# Autodesk Inventor assembly: CanSat
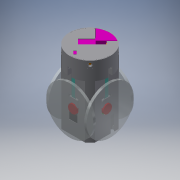
[picture p0: Inventor's stored thumbnail of the model, 180x180]
Saved by Autodesk Inventor 2018 (Build 220112000, 112)
## iProperties
Created: 2017-12-31
Part Number: CanSat
Document SubType Name: Assembly
Designer: suchanek
Author: suchanek
## Documents named in this file (19)
- C:\Users\Suchanek\Programming\CanSat\Schematics\Model\CanSat.iam
- C:\Users\Suchanek\Programming\CanSat\Schematics\Model\Hull.ipt
- C:\Users\Suchanek\Programming\CanSat\Schematics\Model\Arm.ipt
- C:\Users\Suchanek\Programming\CanSat\Schematics\Model\Motor.ipt
- C:\Users\Suchanek\Programming\CanSat\Schematics\Model\Rotor.ipt
- C:\Users\Suchanek\Programming\CanSat\Schematics\Model\Servo.ipt
- C:\Users\Suchanek\Programming\CanSat\Schematics\Model\Spring.ipt
- C:\Users\Suchanek\Programming\CanSat\Schematics\Model\Servo_bit.ipt
- C:\Users\Suchanek\Programming\CanSat\Schematics\Model\Scraper.ipt
- C:\Users\Suchanek\Programming\CanSat\Schematics\Model\Circuit.ipt
- C:\Users\Suchanek\Programming\CanSat\Schematics\Model\Flight_controler.ipt
- C:\Users\Suchanek\Programming\CanSat\Schematics\Model\HGLRC Micro 13A 4in1 BLHeli_S.ipt
- C:\Users\Suchanek\Programming\CanSat\Schematics\Model\SIM808 Module GSM GPRS GPS Breakout Board SIM808 for Arduino Raspberry.ipt
- C:\Users\Suchanek\Programming\CanSat\Schematics\Model\Motor_holder.ipt
- C:\Users\Suchanek\Programming\CanSat\Schematics\Model\Battery.ipt
- C:\Users\Suchanek\Programming\CanSat\Schematics\Model\Hull_bottom.ipt
- C:\Users\Suchanek\Programming\CanSat\Schematics\Model\Camera.ipt
- C:\Users\Suchanek\Programming\CanSat\Schematics\Model\Hull_middle.ipt
- C:\Users\Suchanek\Programming\CanSat\Schematics\Model\Hull_top.ipt
## Components (45 placed, 18 different names)
1. Hull:1 — Slider:2, Rotational:31, Flush:1, Mate:5, Mate:6, Angle:4, Mate:8, Flush:3, Mate:9, Mate:10, Cylindrical:1, Angle:5, Mate:11, Mate:12, Flush:12, Cylindrical:2, Mate:14, Mate:15, Mate:16, Mate:17, Mate:18, Flush:13, Mate:19, Mate:20, Flush:14, Mate:21, Angle:6, Flush:15, Flush:16, Mate:23, Mate:25, Mate:26
2. Servo:1 — Rotational:24, Mate:8, Flush:3, Mate:9
3. Spring:1 — Rigid:6, Rigid:7
4. Servo_bit:1 — Rotational:24, Rigid:6
5. Scraper:1 — Rigid:7
6. Circuit:1 — Mate:21, Angle:6, Flush:15, Mate:24
7. Flight_controler:1 — Cylindrical:1, Angle:5, Mate:11
8. HGLRC Micro 13A 4in1 BLHeli_S:2 — Cylindrical:2, Mate:14, Mate:15
9. SIM808 Module GSM GPRS GPS Breakout Board SIM808 for Arduino Raspberry:1 — Mate:12, Flush:12, Mate:26
10. Hull_bottom:1 — Mate:16, Mate:17, Mate:18
11. Camera:1 — Angle:4, Mate:10, Flush:13
12. Hull_middle:1 — Mate:19, Mate:20, Flush:14
13. Hull_top:1 — Flush:16, Mate:23, Mate:24, Mate:25
14. Battery:2 — Rigid:19, Rigid:20
15. Battery:1 — Rigid:18, Slider:2
16. Battery:3 — Rigid:20, Mate:5
17. Battery:4 — Rigid:18, Rigid:19, Flush:1, Mate:6
18. Battery:5
19. Battery:6
20. Battery:7
21. Battery:8
22. Battery:9
23. Battery:10
24. Battery:11
25. Battery:12
26. Battery:13
27. Battery:14
28. Battery:15
29. Battery:16
30. Arm:1 — Rotational:31, Rigid:21
31. Rotor:2 — Rotational:10
32. Motor:4 — Rotational:10, Rigid:14
33. Motor_holder:2 — Rigid:14, Rigid:21
34. Arm:2
35. Rotor:3
36. Motor:5
37. Motor_holder:3
38. Arm:3
39. Rotor:4
40. Motor:6
41. Motor_holder:4
42. Arm:4
43. Rotor:5
44. Motor:7
45. Motor_holder:5
## Component patterns: (4 elements, first: Battery:2 + Battery:1 + Battery:3 + Battery:4), (4 elements, first: Arm:1 + Rotor:2 + Motor:4 + Motor_holder:2)
## Relationships (42: Mate 19, WeldJoint 7, Flush 7, RevoluteJoint 3, Angle 3, CylindricalJoint 2, TranslationJoint 1)
- Rotational:10 [RevoluteJoint]: Rotor:2 ↔ Motor:4
- Rotational:24 [RevoluteJoint]: Servo:1 ↔ Servo_bit:1
- Rigid:6 [WeldJoint]: Spring:1 ↔ Servo_bit:1
- Rigid:7 [WeldJoint]: Spring:1 ↔ Scraper:1
- Rigid:14 [WeldJoint]: Motor:4 ↔ Motor_holder:2
- Rigid:18 [WeldJoint]: Battery:1 ↔ Battery:4
- Rigid:19 [WeldJoint]: Battery:2 ↔ Battery:4
- Rigid:20 [WeldJoint]: Battery:2 ↔ Battery:3
- Slider:2 [TranslationJoint]: Hull:1 ↔ Battery:1
- Rotational:31 [RevoluteJoint]: Hull:1 ↔ Arm:1
- Flush:1: Hull:1 ↔ Battery:4
- Mate:5: Hull:1 ↔ Battery:3
- Mate:6 (0.25 mm): Hull:1 ↔ Battery:4
- Angle:4 (0 deg): Hull:1 ↔ Camera:1
- Mate:8: Hull:1 ↔ Servo:1
- Flush:3: Hull:1 ↔ Servo:1
- Mate:9: Hull:1 ↔ Servo:1
- Mate:10 (0.1 mm): Hull:1 ↔ Camera:1
- Cylindrical:1: Hull:1 ↔ Flight_controler:1
- Angle:5 (0 deg): Hull:1 ↔ Flight_controler:1
- Mate:11 (-1.5 mm): Hull:1 ↔ Flight_controler:1
- Mate:12: Hull:1 ↔ SIM808 Module GSM GPRS GPS Breakout Board SIM808 for Arduino Raspberry:1
- Flush:12: Hull:1 ↔ SIM808 Module GSM GPRS GPS Breakout Board SIM808 for Arduino Raspberry:1
- Cylindrical:2: Hull:1 ↔ HGLRC Micro 13A 4in1 BLHeli_S:2
- Mate:14: Hull:1 ↔ HGLRC Micro 13A 4in1 BLHeli_S:2
- Mate:15: Hull:1 ↔ HGLRC Micro 13A 4in1 BLHeli_S:2
- Mate:16: Hull:1 ↔ Hull_bottom:1
- Mate:17: Hull:1 ↔ Hull_bottom:1
- Mate:18: Hull:1 ↔ Hull_bottom:1
- Flush:13: Hull:1 ↔ Camera:1
- Rigid:21 [WeldJoint]: Arm:1 ↔ Motor_holder:2
- Mate:19: Hull:1 ↔ Hull_middle:1
- Mate:20: Hull:1 ↔ Hull_middle:1
- Flush:14: Hull:1 ↔ Hull_middle:1
- Mate:21: Hull:1 ↔ Circuit:1
- Angle:6 (0 deg): Hull:1 ↔ Circuit:1
- Flush:15: Hull:1 ↔ Circuit:1
- Flush:16: Hull:1 ↔ Hull_top:1
- Mate:23: Hull:1 ↔ Hull_top:1
- Mate:24: Circuit:1 ↔ Hull_top:1
- Mate:25: Hull:1 ↔ Hull_top:1
- Mate:26: Hull:1 ↔ SIM808 Module GSM GPRS GPS Breakout Board SIM808 for Arduino Raspberry:1
